# Autodesk Inventor assembly: ASY MSC 204 BELLY
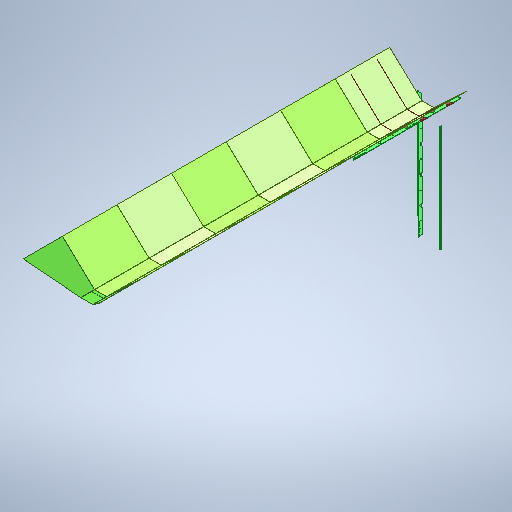
[picture p0: Inventor's stored thumbnail of the model, 512x512]
Saved by Autodesk Inventor 2025 (Build 290162010, 162A)
## iProperties
Created: 2024-07-22
Part Number: ASY MSC 204 BELLY
Document SubType Name: Assembly
Designer: pokla
Author: pokla
## Documents named in this file (5)
- C:\Users\user\YandexDisk\домашниий пк\Inventor\Manturovo\Manturovo_Se-clar\ASY MSC 204 BELLY.iam
- C:\Users\user\YandexDisk\домашниий пк\Inventor\Manturovo\Manturovo_Se-clar\MSC 041 sheet belly main.ipt
- C:\Users\user\YandexDisk\домашниий пк\Inventor\Manturovo\Manturovo_Se-clar\MSC 042 sheet belly-neck.ipt
- C:\Users\user\YandexDisk\домашниий пк\Inventor\Manturovo\Manturovo_Se-clar\MSC 067 stringer board belly.ipt
- C:\Users\user\YandexDisk\домашниий пк\Inventor\Manturovo\Manturovo_Se-clar\MSC 053 rib belly.ipt
## Components (19 placed, 4 different names)
1. MSC 041 sheet belly main.ipt:1
2. MSC 041 sheet belly main.ipt:2
3. MSC 041 sheet belly main.ipt:3
4. MSC 042 sheet belly-neck.ipt:1
5. MSC 041 sheet belly main.ipt:4
6. MSC 041 sheet belly main.ipt:5
7. MSC 041 sheet belly main.ipt:6 — Mate:4, Mate:5, Mate:6, Mate:7, Flush:1, Mate:9, Mate:10
8. MSC 067 stringer board belly.ipt:4
9. MSC 067 stringer board belly.ipt:3
10. MSC 067 stringer board belly.ipt:1
11. MSC 067 stringer board belly.ipt:2
12. MSC 053 rib belly.ipt:2 — Mate:4, Mate:5, Mate:8
13. MSC 053 rib belly.ipt:1 — Mate:6, Mate:7, Mate:8, Rigid:17
14. MSC 053 rib belly.ipt:4 — Rigid:17
15. MSC 053 rib belly.ipt:3 — Rigid:18
16. MSC 067 stringer board belly.ipt:5
17. MSC 067 stringer board belly.ipt:6
18. MSC 067 stringer board belly.ipt:8
19. MSC 067 stringer board belly.ipt:7 — Rigid:18
## Relationships (21: WeldJoint 13, Mate 7, Flush 1)
- [WeldJoint]: MSC 041 sheet belly main.ipt:1 ↔ MSC 041 sheet belly main.ipt:2
- [WeldJoint]: MSC 041 sheet belly main.ipt:1 ↔ MSC 041 sheet belly main.ipt:3
- [WeldJoint]: MSC 041 sheet belly main.ipt:4 ↔ MSC 041 sheet belly main.ipt:5
- [WeldJoint]: MSC 041 sheet belly main.ipt:3 ↔ MSC 041 sheet belly main.ipt:4
- [WeldJoint]: MSC 042 sheet belly-neck.ipt:1 ↔ MSC 041 sheet belly main.ipt:5
- [WeldJoint]: MSC 041 sheet belly main.ipt:2 ↔ MSC 041 sheet belly main.ipt:6
- [WeldJoint] (-50 mm): MSC 053 rib belly.ipt:4 ↔ MSC 053 rib belly.ipt:3
- [WeldJoint]: MSC 067 stringer board belly.ipt:2 ↔ MSC 067 stringer board belly.ipt:8
- [WeldJoint]: MSC 067 stringer board belly.ipt:1 ↔ MSC 067 stringer board belly.ipt:7
- [WeldJoint]: MSC 067 stringer board belly.ipt:3 ↔ MSC 067 stringer board belly.ipt:6
- [WeldJoint]: MSC 067 stringer board belly.ipt:4 ↔ MSC 067 stringer board belly.ipt:5
- Mate:4: MSC 041 sheet belly main.ipt:6 ↔ MSC 053 rib belly.ipt:2
- Mate:5: MSC 041 sheet belly main.ipt:6 ↔ MSC 053 rib belly.ipt:2
- Mate:6: MSC 041 sheet belly main.ipt:6 ↔ MSC 053 rib belly.ipt:1
- Mate:7: MSC 041 sheet belly main.ipt:6 ↔ MSC 053 rib belly.ipt:1
- Mate:8: MSC 053 rib belly.ipt:2 ↔ MSC 053 rib belly.ipt:1
- Flush:1: MSC 041 sheet belly main.ipt:6
- Mate:9: MSC 041 sheet belly main.ipt:6
- Mate:10: MSC 041 sheet belly main.ipt:6
- Rigid:17 [WeldJoint] (480 mm): MSC 053 rib belly.ipt:1 ↔ MSC 053 rib belly.ipt:4
- Rigid:18 [WeldJoint]: MSC 053 rib belly.ipt:3 ↔ MSC 067 stringer board belly.ipt:7
